# Autodesk Inventor assembly: Assembly
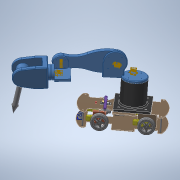
[picture p0: Inventor's stored thumbnail of the model, 180x180]
Saved by Autodesk Inventor 2021 (Build 250183000, 183)
## iProperties
Created: 2021-07-13
Part Number: Assembly
Document SubType Name: Assembly
Designer: Administrator
Title: Assembly v65
Author: Administrator
## Documents named in this file (15)
- C:\Users\ASUS\Desktop\robo arm\Assembly.iam
- C:\Users\ASUS\Desktop\robo arm\Base v7.ipt
- C:\Users\ASUS\Desktop\robo arm\Motor mount 1 v7.ipt
- C:\Users\ASUS\Desktop\robo arm\servo5 v1.iam
- C:\Users\ASUS\Desktop\robo arm\Link v2.ipt
- C:\Users\ASUS\Desktop\robo arm\servo5 v1_1.iam
- C:\Users\ASUS\Desktop\robo arm\Motor mount 2 v3.ipt
- C:\Users\ASUS\Desktop\robo arm\servo5 v1_2.iam
- C:\Users\ASUS\Desktop\robo arm\servo5 v1_3.iam
- C:\Users\ASUS\Desktop\robo arm\Robotic arm gripper v4.ipt
- C:\Users\ASUS\Desktop\robo arm\Auxilary component v4.ipt
- C:\Users\ASUS\Desktop\robo arm\Gripper v2.ipt
- C:\Users\ASUS\Desktop\robo arm\Marker v1.ipt
- C:\Users\ASUS\Desktop\3d model\CARRO ROBÓTICO.iam
- C:\Users\ASUS\Desktop\robotic arm\5mm LED.ipt
## Components (14 placed, 11 different names)
1. Base v7:1 — Flush:1, Rotational:10
2. Motor mount 1 v7:1 — Rotational:2, Rotational:8, Rotational:9, Rotational:10
3. servo5 v1:1 [sub-assembly] — Rotational:2
4. Link v2:1 — Rigid:4, Rotational:8
5. servo5 v1:2 [sub-assembly] — Rotational:9
6. Motor mount 2 v3:1 — Rigid:4, Rotational:4, Rotational:5, Rigid:1
7. servo5 v1:3 [sub-assembly] — Rigid:1
8. servo5 v1:4 [sub-assembly] — Rotational:5
9. Robotic arm gripper v4:1 — Rotational:4, Rotational:6
10. Auxilary component v4:2 — Rotational:6, Rotational:7
11. Gripper v2:1 — Rigid:5, Rotational:7
12. Marker v1:1 — Rigid:5
13. CARRO ROBÓTICO:1 [sub-assembly] — Flush:1, Mate:1
14. 5mm LED:2 — Mate:1
## Relationships (13: RevoluteJoint 8, WeldJoint 3, Flush 1, Mate 1)
- Rigid:5 [WeldJoint]: Gripper v2:1 ↔ Marker v1:1
- Flush:1: Base v7:1 ↔ CARRO ROBÓTICO:1
- Rotational:2 [RevoluteJoint]: Motor mount 1 v7:1 ↔ servo5 v1:1
- Rigid:4 [WeldJoint]: Link v2:1 ↔ Motor mount 2 v3:1
- Rotational:4 [RevoluteJoint]: Motor mount 2 v3:1 ↔ Robotic arm gripper v4:1
- Rotational:5 [RevoluteJoint]: Motor mount 2 v3:1 ↔ servo5 v1:4
- Rigid:1 [WeldJoint]: Motor mount 2 v3:1 ↔ servo5 v1:3
- Rotational:6 [RevoluteJoint]: Robotic arm gripper v4:1 ↔ Auxilary component v4:2
- Rotational:7 [RevoluteJoint]: Auxilary component v4:2 ↔ Gripper v2:1
- Rotational:8 [RevoluteJoint]: Motor mount 1 v7:1 ↔ Link v2:1
- Rotational:9 [RevoluteJoint]: Motor mount 1 v7:1 ↔ servo5 v1:2
- Rotational:10 [RevoluteJoint]: Base v7:1 ↔ Motor mount 1 v7:1
- Mate:1: CARRO ROBÓTICO:1 ↔ 5mm LED:2
